# Autodesk Inventor assembly: calosc
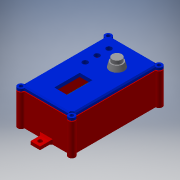
[picture p0: Inventor's stored thumbnail of the model, 180x180]
Saved by Autodesk Inventor 2019 (Build 230136000, 136)
## iProperties
Created: 2019-09-16
Part Number: calosc
Material: Ogólny
Document SubType Name: Assembly
Designer: mikol
Author: mikol
## Documents named in this file (5)
- C:\Users\mikol\Desktop\Projekty\Pomiar_poziomu_wody\baza\projekt_obudowy\calosc_V2.iam
- C:\Users\mikol\Desktop\Projekty\Pomiar_poziomu_wody\baza\projekt_obudowy\PCB.ipt
- C:\Users\mikol\Desktop\Projekty\Pomiar_poziomu_wody\baza\projekt_obudowy\przycisk.ipt
- C:\Users\mikol\Desktop\Projekty\Pomiar_poziomu_wody\baza\projekt_obudowy\gora_V2.ipt
- C:\Users\mikol\Desktop\Projekty\Pomiar_poziomu_wody\baza\projekt_obudowy\Podstawa_V2.ipt
## Components (4 placed, 4 different names)
1. PCB:1 — Rigid:4
2. przycisk:1 — Rigid:3
3. gora_V2:1 — Rigid:3, Rigid:5
4. Podstawa_V2:2 — Rigid:4, Rigid:5
## Relationships (3: WeldJoint 3)
- Rigid:3 [WeldJoint]: przycisk:1 ↔ gora_V2:1
- Rigid:4 [WeldJoint]: PCB:1 ↔ Podstawa_V2:2
- Rigid:5 [WeldJoint] (-1 mm): gora_V2:1 ↔ Podstawa_V2:2
